# Autodesk Inventor assembly: kneader assembly
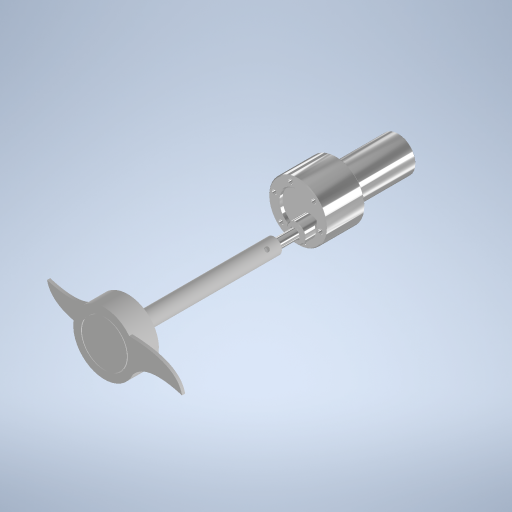
[picture p0: Inventor's stored thumbnail of the model, 512x512]
Saved by Autodesk Inventor 2023 (Build 270158000, 158)
## iProperties
Created: 2022-05-20
Part Number: kneader assembly
Document SubType Name: Assembly
Designer: techv
Author: techv
## Documents named in this file (4)
- D:\Projects\P_Baker Bot\Design\kneader assembly - v2.iam
- D:\Projects\P_Baker Bot\Design\JHONSON 12V DC GEARED MOTOR.ipt
- D:\Projects\P_Baker Bot\Design\kneading blade - v2.ipt
- D:\Projects\P_Baker Bot\Design\kneading shaft - v2.ipt
## Components (3 placed, 3 different names)
1. JHONSON 12V DC GEARED MOTOR:1 — Mate:1, Mate:5
2. kneading blade - v2:1 — Mate:3, Mate:4
3. kneading shaft - v2:1 — Mate:1, Mate:3, Mate:4, Mate:5
## Relationships (4: Mate 4)
- Mate:1: JHONSON 12V DC GEARED MOTOR:1 ↔ kneading shaft - v2:1
- Mate:3: kneading blade - v2:1 ↔ kneading shaft - v2:1
- Mate:4: kneading blade - v2:1 ↔ kneading shaft - v2:1
- Mate:5: JHONSON 12V DC GEARED MOTOR:1 ↔ kneading shaft - v2:1
